# Autodesk Inventor assembly: Assembly1
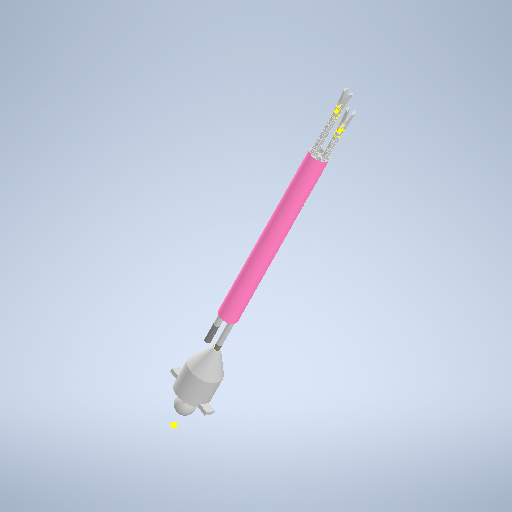
[picture p0: Inventor's stored thumbnail of the model, 512x512]
Saved by Autodesk Inventor 2025.2 (Build 292293000, 293)
## iProperties
Created: 2025-04-30
Part Number: Assembly1
Document SubType Name: Assembly
Designer: avnr2
Author: avnr2
## Documents named in this file (6)
- C:\Users\avnr2\OneDrive\Desktop\CAD- desgin tool\Assembly1.iam
- C:\Users\avnr2\OneDrive\Desktop\project\tool 1.1.ipt
- C:\Users\avnr2\OneDrive\Desktop\project\outer casing.ipt
- C:\Users\avnr2\OneDrive\Desktop\CAD- desgin tool\Joy stick part 2.ipt
- C:\Users\avnr2\OneDrive\Desktop\CAD- desgin tool\joy stick part 1.ipt
- C:\Users\avnr2\OneDrive\Desktop\CAD- desgin tool\Part3.ipt
## Components (6 placed, 5 different names)
1. tool 1.1:1 — Mate:2, Mate:3, Mate:4
2. tool 1.1:2 — Mate:1
3. outer casing:1 — Mate:1, Mate:2
4. Joy stick part 2:1 — Mate:3, Mate:5
5. joy stick part 1:1 — Mate:4
6. Part3:1 — Mate:5
## Relationships (5: Mate 5)
- Mate:1: tool 1.1:2 ↔ outer casing:1
- Mate:2: tool 1.1:1 ↔ outer casing:1
- Mate:3: tool 1.1:1 ↔ Joy stick part 2:1
- Mate:4: tool 1.1:1 ↔ joy stick part 1:1
- Mate:5: Joy stick part 2:1 ↔ Part3:1
